# Autodesk Inventor assembly: Roller_Bracket
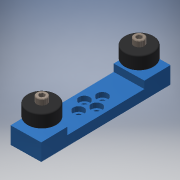
[picture p0: Inventor's stored thumbnail of the model, 180x180]
Saved by Autodesk Inventor 2019.4 (Build 234330000, 330)
## iProperties
Created: 2021-02-01
Part Number: Roller_Bracket
Document SubType Name: Assembly
Designer: Jorian Brusind
Mass: 44.0669 g
Surface Area: 169.812 cm^2
Volume: 42.4218 cm^3
Density: 1.03878 g/cm^3
Author: Jorian Brusind
## Documents named in this file (4)
- C:\Users\Jorian Brusind\Documents\GitHub\PersonalProjects\HyperRail\Inventor Files\Roller_Bracket.iam
- C:\Users\Jorian Brusind\Documents\GitHub\PersonalProjects\HyperRail\Inventor Files\Back_Bracket.ipt
- C:\Users\Jorian Brusind\Documents\GitHub\PersonalProjects\HyperRail\Inventor Files\11mm_BearingWheel.ipt
- C:\Users\Jorian Brusind\Documents\GitHub\PersonalProjects\Inventor Projects\Useful models\Metric bolt\Bolt M5 20mm.ipt
## Components (5 placed, 3 different names)
1. Back_Bracket:1 — Mate:1, Mate:3, Mate:5, Mate:7
2. 11mm_BearingWheel:1 — Mate:1, Mate:2, Mate:3, Mate:4
3. 11mm_BearingWheel:2 — Mate:5, Mate:6, Mate:7, Mate:8
4. Bolt M5 20mm:1 — Mate:6, Mate:8
5. Bolt M5 20mm:2 — Mate:2, Mate:4
## Relationships (8: Mate 8)
- Mate:1: Back_Bracket:1 ↔ 11mm_BearingWheel:1
- Mate:2: 11mm_BearingWheel:1 ↔ Bolt M5 20mm:2
- Mate:3 (5 mm): Back_Bracket:1 ↔ 11mm_BearingWheel:1
- Mate:4: 11mm_BearingWheel:1 ↔ Bolt M5 20mm:2
- Mate:5: Back_Bracket:1 ↔ 11mm_BearingWheel:2
- Mate:6: 11mm_BearingWheel:2 ↔ Bolt M5 20mm:1
- Mate:7 (5 mm): Back_Bracket:1 ↔ 11mm_BearingWheel:2
- Mate:8: 11mm_BearingWheel:2 ↔ Bolt M5 20mm:1
